# Autodesk Inventor assembly: hand
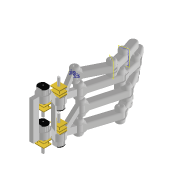
[picture p0: Inventor's stored thumbnail of the model, 180x180]
Saved by Autodesk Inventor 2020.2 (Build 242310000, 310)
## iProperties
Created: 2020-04-08
Part Number: hand
Document SubType Name: Assembly
Designer: Bardo91
thread_hole: 2.500 mm
Author: Bardo91
## Documents named in this file (15)
- D:\programming\bioarm\hardware\hand\hand.iam
- D:\programming\bioarm\hardware\hand\pinky_f1.ipt
- D:\programming\bioarm\hardware\hand\pinky_f2.ipt
- D:\programming\bioarm\hardware\hand\pinky_f3.ipt
- D:\programming\bioarm\hardware\hand\ring_f1.ipt
- D:\programming\bioarm\hardware\hand\ring_f2.ipt
- D:\programming\bioarm\hardware\hand\ring_f3.ipt
- D:\programming\bioarm\hardware\hand\middle_f1.ipt
- D:\programming\bioarm\hardware\hand\middle_f2.ipt
- D:\programming\bioarm\hardware\hand\middle_f3.ipt
- D:\programming\bioarm\hardware\hand\index_f1.ipt
- D:\programming\bioarm\hardware\hand\index_f2.ipt
- D:\programming\bioarm\hardware\hand\index_f3.ipt
- D:\programming\bioarm\hardware\hand\base_hand.ipt
- D:\programming\bioarm\hardware\hand\motor_dc_6v_30rpm.ipt
## Components (17 placed, 14 different names)
1. base_hand:1 — Flush:9, Flush:10, Flush:11, Flush:12, Mate:9, Mate:10, Mate:11, Mate:12, Mate:13, Mate:14, Mate:15, Mate:16, Mate:17, Mate:18, Mate:19, Mate:20, Mate:21, Mate:22, Mate:23, Mate:24
2. motor_dc_6v_30rpm:1 — Mate:14, Mate:19, Mate:24
3. motor_dc_6v_30rpm:2 — Mate:16, Mate:17, Mate:18
4. motor_dc_6v_30rpm:3 — Mate:13, Mate:20, Mate:23
5. motor_dc_6v_30rpm:4 — Mate:15, Mate:21, Mate:22
6. pinky_f1:1 — Mate:1, Flush:1, Flush:9, Mate:12
7. pinky_f2:1 — Mate:1, Flush:1, Flush:2, Mate:2
8. pinky_f3:1 — Flush:2, Mate:2
9. ring_f1:1 — Flush:3, Mate:3, Flush:10, Mate:11
10. ring_f2:1 — Flush:3, Flush:4, Mate:3, Mate:4
11. ring_f3:1 — Flush:4, Mate:4
12. middle_f1:1 — Flush:5, Mate:6, Flush:11, Mate:10
13. middle_f2:1 — Flush:5, Flush:6, Mate:5, Mate:6
14. middle_f3:1 — Flush:6, Mate:5
15. index_f1:1 — Flush:7, Mate:8, Flush:12, Mate:9
16. index_f2:1 — Flush:7, Flush:8, Mate:7, Mate:8
17. index_f3:1 — Flush:8, Mate:7
## Relationships (36: Mate 24, Flush 12)
- Mate:1: pinky_f1:1 ↔ pinky_f2:1
- Flush:1: pinky_f1:1 ↔ pinky_f2:1
- Flush:2: pinky_f2:1 ↔ pinky_f3:1
- Mate:2: pinky_f2:1 ↔ pinky_f3:1
- Flush:3: ring_f1:1 ↔ ring_f2:1
- Flush:4: ring_f2:1 ↔ ring_f3:1
- Mate:3: ring_f1:1 ↔ ring_f2:1
- Mate:4: ring_f2:1 ↔ ring_f3:1
- Flush:5: middle_f1:1 ↔ middle_f2:1
- Flush:6: middle_f2:1 ↔ middle_f3:1
- Mate:5: middle_f2:1 ↔ middle_f3:1
- Mate:6: middle_f1:1 ↔ middle_f2:1
- Flush:7: index_f1:1 ↔ index_f2:1
- Flush:8: index_f2:1 ↔ index_f3:1
- Mate:7: index_f2:1 ↔ index_f3:1
- Mate:8: index_f1:1 ↔ index_f2:1
- Flush:9: base_hand:1 ↔ pinky_f1:1
- Flush:10: base_hand:1 ↔ ring_f1:1
- Flush:11: base_hand:1 ↔ middle_f1:1
- Flush:12: base_hand:1 ↔ index_f1:1
- Mate:9: base_hand:1 ↔ index_f1:1
- Mate:10: base_hand:1 ↔ middle_f1:1
- Mate:11: base_hand:1 ↔ ring_f1:1
- Mate:12: base_hand:1 ↔ pinky_f1:1
- Mate:13: base_hand:1 ↔ motor_dc_6v_30rpm:3
- Mate:14: base_hand:1 ↔ motor_dc_6v_30rpm:1
- Mate:15: base_hand:1 ↔ motor_dc_6v_30rpm:4
- Mate:16: base_hand:1 ↔ motor_dc_6v_30rpm:2
- Mate:17: base_hand:1 ↔ motor_dc_6v_30rpm:2
- Mate:18: base_hand:1 ↔ motor_dc_6v_30rpm:2
- Mate:19: base_hand:1 ↔ motor_dc_6v_30rpm:1
- Mate:20: base_hand:1 ↔ motor_dc_6v_30rpm:3
- Mate:21: base_hand:1 ↔ motor_dc_6v_30rpm:4
- Mate:22: base_hand:1 ↔ motor_dc_6v_30rpm:4
- Mate:23: base_hand:1 ↔ motor_dc_6v_30rpm:3
- Mate:24: base_hand:1 ↔ motor_dc_6v_30rpm:1
## Named parameters: thread_hole = 2.5 mm
